# Autodesk Inventor assembly: 100.001.01_Lernfabrik
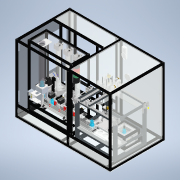
[picture p0: Inventor's stored thumbnail of the model, 180x180]
Saved by Autodesk Inventor 2022 (Build 260153000, 153)
## iProperties
Created: 2021-12-04
Part Number: 100.001.01_Lernfabrik
Document SubType Name: Assembly
Designer: Sebastian Seewald
Author: Sebastian Seewald
## Documents named in this file (5)
- C:\Users\kaebi\OneDrive - mci4me.at\03_MCI Master\4.Semester_SS2022\Masterarbeit\2_WorkDir\2_CadTeachingFactory\100.001.01_Lernfabrik.iam
- C:\Users\kaebi\OneDrive - mci4me.at\03_MCI Master\4.Semester_SS2022\Masterarbeit\2_WorkDir\2_CadTeachingFactory\201.001.01_ZB_Rahmen_GBG.iam
- C:\Users\kaebi\OneDrive - mci4me.at\03_MCI Master\4.Semester_SS2022\Masterarbeit\2_WorkDir\2_CadTeachingFactory\203.001.01_ZB_Modul.iam
- C:\Users\kaebi\OneDrive - mci4me.at\03_MCI Master\4.Semester_SS2022\Masterarbeit\2_WorkDir\2_CadTeachingFactory\500.001.01_HMI_Pannel.ipt
- C:\Users\kaebi\OneDrive - mci4me.at\03_MCI Master\4.Semester_SS2022\Masterarbeit\2_WorkDir\2_CadTeachingFactory\Kartesischer_Roboter_Modul.iam
## Components (4 placed, 4 different names)
1. 201.001.01_ZB_Rahmen_GBG:1 [sub-assembly] — Passend:1, Fluchtend:1, Fluchtend:2, Passend:5, Passend:6, Passend:8, Mate:9, Mate:10, Flush:4
2. 203.001.01_ZB_Modul:1 [sub-assembly] — Passend:1, Fluchtend:1, Passend:8
3. 500.001.01_HMI_Pannel:1 — Fluchtend:2, Passend:5, Passend:6
4. Kartesischer_Roboter_Modul:1 [sub-assembly] — Mate:9, Mate:10, Flush:4
## Relationships (9: Mate 6, Flush 3)
- Passend:1 [Mate]: 201.001.01_ZB_Rahmen_GBG:1 ↔ 203.001.01_ZB_Modul:1
- Fluchtend:1 [Flush]: 201.001.01_ZB_Rahmen_GBG:1 ↔ 203.001.01_ZB_Modul:1
- Fluchtend:2 [Flush]: 201.001.01_ZB_Rahmen_GBG:1 ↔ 500.001.01_HMI_Pannel:1
- Passend:5 [Mate] (30 mm): 201.001.01_ZB_Rahmen_GBG:1 ↔ 500.001.01_HMI_Pannel:1
- Passend:6 [Mate] (250 mm): 201.001.01_ZB_Rahmen_GBG:1 ↔ 500.001.01_HMI_Pannel:1
- Passend:8 [Mate] (20 mm): 201.001.01_ZB_Rahmen_GBG:1 ↔ 203.001.01_ZB_Modul:1
- Mate:9: 201.001.01_ZB_Rahmen_GBG:1 ↔ Kartesischer_Roboter_Modul:1
- Mate:10 (85 mm): 201.001.01_ZB_Rahmen_GBG:1 ↔ Kartesischer_Roboter_Modul:1
- Flush:4: 201.001.01_ZB_Rahmen_GBG:1 ↔ Kartesischer_Roboter_Modul:1
